# Autodesk Inventor assembly: Frezowanie_male No.2
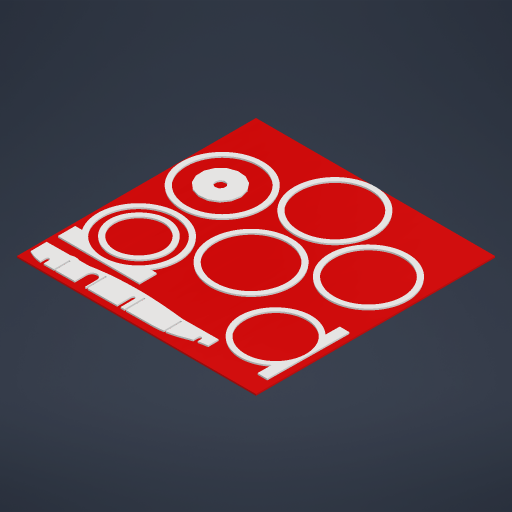
[picture p0: Inventor's stored thumbnail of the model, 512x512]
Saved by Autodesk Inventor 2023 (Build 270158000, 158)
## iProperties
Created: 2023-04-06
Part Number: Frezowanie_male No.2
Document SubType Name: Assembly
Designer: szykr
Author: szykr
## Documents named in this file (11)
- D:\Folder Instalacyjny\GitHub Pliki\Solaris\new model\Frez\Frezowanie_male No.2.iam
- D:\Folder Instalacyjny\GitHub Pliki\Solaris\new model\Frez\Laminat235x235.ipt
- D:\Folder Instalacyjny\GitHub Pliki\Solaris\new model\Frez\Troche Mniejsze(2-31)\Solid7.ipt
- D:\Folder Instalacyjny\GitHub Pliki\Solaris\new model\Frez\Troche Mniejsze(2-31)\Solid8.ipt
- D:\Folder Instalacyjny\GitHub Pliki\Solaris\new model\Frez\Troche Mniejsze(2-31)\Solid9.ipt
- D:\Folder Instalacyjny\GitHub Pliki\Solaris\new model\Frez\Troche Mniejsze(2-31)\Solid10.ipt
- D:\Folder Instalacyjny\GitHub Pliki\Solaris\new model\Frez\Troche Mniejsze(2-31)\Solid11.ipt
- D:\Folder Instalacyjny\GitHub Pliki\Solaris\new model\Frez\Troche Mniejsze(2-31)\Solid12.ipt
- D:\Folder Instalacyjny\GitHub Pliki\Solaris\new model\Frez\Troche Mniejsze(2-31)\Solid13.ipt
- D:\Folder Instalacyjny\GitHub Pliki\Solaris\new model\Frez\Troche Mniejsze(2-31)\Solid14.ipt
- D:\Folder Instalacyjny\GitHub Pliki\Solaris\new model\Frez\Troche Mniejsze(2-31)\Solid31.ipt
## Components (10 placed, 10 different names)
1. Laminat235x235:1 — Mate:1, Mate:2, Mate:3, Mate:4, Mate:5, Mate:6, Mate:7, Mate:8, Mate:9
2. Solid7:1 — Mate:1
3. Solid8:1 — Mate:2
4. Solid9:1 — Mate:3
5. Solid10:1 — Mate:4
6. Solid11:1 — Mate:5
7. Solid12:1 — Mate:6
8. Solid13:1 — Mate:7
9. Solid14:1 — Mate:8
10. Solid31:1 — Mate:9
## Relationships (9: Mate 9)
- Mate:1: Laminat235x235:1 ↔ Solid7:1
- Mate:2: Laminat235x235:1 ↔ Solid8:1
- Mate:3: Laminat235x235:1 ↔ Solid9:1
- Mate:4: Laminat235x235:1 ↔ Solid10:1
- Mate:5: Laminat235x235:1 ↔ Solid11:1
- Mate:6: Laminat235x235:1 ↔ Solid12:1
- Mate:7: Laminat235x235:1 ↔ Solid13:1
- Mate:8: Laminat235x235:1 ↔ Solid14:1
- Mate:9: Laminat235x235:1 ↔ Solid31:1
